# Autodesk Inventor assembly: pcb_assembly
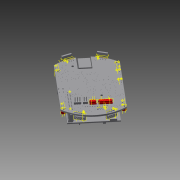
[picture p0: Inventor's stored thumbnail of the model, 180x180]
Saved by Autodesk Inventor 2014 (Build 180170000, 170)
## iProperties
Created: 2013-08-25
Part Number: pcb_assembly
Document SubType Name: Assembly
Designer: Felix
Author: Felix
## Documents named in this file (4)
- C:\Users\Felix\Desktop\Beep\Hardware\3D-CAD\parts\electronic\pcb_assembly.iam
- C:\Users\Felix\Desktop\Beep\Hardware\3D-CAD\parts\electronic\BEEP\beep_main_assembled.iam
- C:\Users\Felix\Desktop\Beep\Hardware\3D-CAD\parts\electronic\RaspberryPi\RaspberryPi.iam
- C:\Users\Felix\Desktop\Beep\Hardware\3D-CAD\parts\electronic\BEEP\beep_rgb_ir_assembled.iam
## Components (4 placed, 3 different names)
1. beep_main_assembled:1 [sub-assembly] — Passend:2, Passend:4, Passend:6, Passend:7, Passend:8, Passend:9, Passend:10
2. RaspberryPi:1 [sub-assembly] — Passend:2
3. beep_rgb_ir_assembled:1 [sub-assembly] — Passend:4, Passend:6, Passend:7
4. beep_rgb_ir_assembled:2 [sub-assembly] — Passend:8, Passend:9, Passend:10
## Relationships (7: Mate 7)
- Passend:2 [Mate]: beep_main_assembled:1 ↔ RaspberryPi:1
- Passend:4 [Mate]: beep_main_assembled:1 ↔ beep_rgb_ir_assembled:1
- Passend:6 [Mate]: beep_main_assembled:1 ↔ beep_rgb_ir_assembled:1
- Passend:7 [Mate]: beep_main_assembled:1 ↔ beep_rgb_ir_assembled:1
- Passend:8 [Mate]: beep_main_assembled:1 ↔ beep_rgb_ir_assembled:2
- Passend:9 [Mate]: beep_main_assembled:1 ↔ beep_rgb_ir_assembled:2
- Passend:10 [Mate]: beep_main_assembled:1 ↔ beep_rgb_ir_assembled:2
